# Autodesk Inventor assembly: V2 - Full Assembly
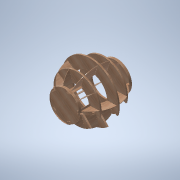
[picture p0: Inventor's stored thumbnail of the model, 180x180]
Saved by Autodesk Inventor 2021 (Build 250183000, 183)
## iProperties
Created: 2020-07-30
Part Number: V2 - Full Assembly
Document SubType Name: Assembly
Designer: Dan Wikman
Author: Dan Wikman
## Documents named in this file (17)
- C:\Users\danny\OneDrive\University Life\2020, Semester 1\METR4900 Honours Thesis\PROTOTYPE V2\V2 - Full Assembly.iam
- C:\Users\danny\OneDrive\University Life\2020, Semester 1\METR4900 Honours Thesis\PROTOTYPE V2\Base - V2.ipt
- C:\Users\danny\OneDrive\University Life\2020, Semester 1\METR4900 Honours Thesis\PROTOTYPE V2\Vertical Support Assembly.iam
- C:\Users\danny\OneDrive\University Life\2020, Semester 1\METR4900 Honours Thesis\PROTOTYPE V2\Support A1 - V2.ipt
- C:\Users\danny\OneDrive\University Life\2020, Semester 1\METR4900 Honours Thesis\PROTOTYPE V2\Level 1 Support Ends.ipt
- C:\Users\danny\OneDrive\University Life\2020, Semester 1\METR4900 Honours Thesis\PROTOTYPE V2\Level 1 Support Mid.ipt
- C:\Users\danny\OneDrive\University Life\2020, Semester 1\METR4900 Honours Thesis\PROTOTYPE V2\Level 1 Ring Assembly.iam
- C:\Users\danny\OneDrive\University Life\2020, Semester 1\METR4900 Honours Thesis\PROTOTYPE V2\Level 3 Assembly.iam
- C:\Users\danny\OneDrive\University Life\2020, Semester 1\METR4900 Honours Thesis\PROTOTYPE V2\Level 2 Ring Assembly.iam
- C:\Users\danny\OneDrive\University Life\2020, Semester 1\METR4900 Honours Thesis\PROTOTYPE V2\Roof - V2.ipt
- C:\Users\danny\OneDrive\University Life\2020, Semester 1\METR4900 Honours Thesis\PROTOTYPE V2\Level 2 Edge Banding.ipt
- C:\Users\danny\OneDrive\University Life\2020, Semester 1\METR4900 Honours Thesis\PROTOTYPE V2\Level 1 Edge Banding.ipt
- C:\Users\danny\OneDrive\University Life\2020, Semester 1\METR4900 Honours Thesis\PROTOTYPE V2\Roof Banding.ipt
- C:\Users\danny\OneDrive\University Life\2020, Semester 1\METR4900 Honours Thesis\PROTOTYPE V2\Floor Banding.ipt
- C:\Users\danny\OneDrive\University Life\2020, Semester 1\METR4900 Honours Thesis\PROTOTYPE V2\Wedge Assembly.iam
- C:\Users\danny\OneDrive\University Life\2020, Semester 1\METR4900 Honours Thesis\PROTOTYPE V2\Feet - V2.ipt
- C:\Users\danny\OneDrive\University Life\2020, Semester 1\METR4900 Honours Thesis\PROTOTYPE V2\Level 3 Edge Banding.ipt
## Components (47 placed, 16 different names)
1. Base - V2:1 — Mate:3, Mate:7, Mate:8, Mate:9, Mate:17, Mate:18, Mate:20, Mate:21, Mate:22, Mate:25, Mate:55, Mate:56, Mate:57, Mate:58, Mate:60
2. Level 1 Support Ends:1 — Mate:16, Mate:17, Mate:18
3. Level 1 Support Ends:2 — Mate:19, Mate:20, Mate:21
4. Level 1 Ring Assembly:1 [sub-assembly] — Mate:31, Mate:32, Mate:33, Mate:47, Mate:48
5. Level 2 Ring Assembly:1 [sub-assembly] — Mate:38, Mate:43, Mate:44, Mate:45, Mate:46, Flush:1
6. Level 3 Assembly:2 [sub-assembly] — Mate:34, Mate:63, Mate:64, Mate:65, Mate:66
7. Roof - V2:1 — Mate:40, Mate:41, Mate:42, Mate:53
8. Level 2 Edge Banding:1 — Mate:45, Mate:46, Flush:1
9. Level 1 Edge Banding:1 — Mate:47, Mate:48, Mate:49
10. Roof Banding:1 — Mate:53, Flush:2
11. Floor Banding:1 — Mate:57, Flush:3
12. Level 3 Edge Banding:1 — Mate:65, Mate:66, Mate:67
13. Vertical Support Assembly:1 [sub-assembly] — Mate:3, Mate:32, Mate:34, Mate:38, Mate:41, Mate:42, Mate:43, Mate:44, Mate:55, Mate:56, Mate:63, Mate:64
14. Vertical Support Assembly:2 [sub-assembly]
15. Vertical Support Assembly:3 [sub-assembly] — Mate:16, Mate:33, Mate:49, Flush:2, Flush:3, Mate:59, Flush:4, Mate:61, Mate:62
16. Vertical Support Assembly:4 [sub-assembly] — Mate:19, Mate:31
17. Vertical Support Assembly:5 [sub-assembly] — Mate:23, Mate:24, Mate:26, Mate:27, Mate:40, Mate:67
18. Support A1 - V2:1 — Mate:7, Mate:9
19. Support A1 - V2:2 — Mate:8
20. Support A1 - V2:3
21. Support A1 - V2:4
22. Level 1 Support Mid:1 — Mate:22, Mate:23, Mate:24
23. Level 1 Support Mid:2 — Mate:25, Mate:26, Mate:27
24. Level 1 Support Mid:3
25. Level 1 Support Mid:4
26. Level 1 Support Mid:5
27. Level 1 Support Mid:6
28. Wedge Assembly:1 [sub-assembly] — Mate:58, Mate:59, Flush:4
29. Wedge Assembly:2 [sub-assembly]
30. Wedge Assembly:3 [sub-assembly]
31. Wedge Assembly:4 [sub-assembly]
32. Wedge Assembly:5 [sub-assembly]
33. Feet - V2:1 — Mate:60, Mate:61, Mate:62
34. Feet - V2:2
35. Feet - V2:3
36. Feet - V2:4
37. Feet - V2:5
38. Feet - V2:6
39. Feet - V2:7
40. Feet - V2:8
41. Feet - V2:9
42. Feet - V2:10
43. Feet - V2:11
44. Feet - V2:12
45. Feet - V2:13
46. Feet - V2:14
47. Feet - V2:15
## Component patterns: (5 elements, first: Vertical Support Assembly:1), (4 elements, first: Support A1 - V2:1), (3 elements, first: Level 1 Support Mid:1 + Level 1 Support Mid:2), (5 elements, first: Wedge Assembly:1), (5 elements), (3 elements, first: Feet - V2:1), Component Pattern 5:2 (3 elements), Component Pattern 5:3 (3 elements), Component Pattern 5:4 (3 elements), Component Pattern 5:5 (3 elements)
## Relationships (49: Mate 45, Flush 4)
- Mate:3 (0.25 mm): Base - V2:1 ↔ Vertical Support Assembly:1
- Mate:7 (0.25 mm): Base - V2:1 ↔ Support A1 - V2:1
- Mate:8: Base - V2:1 ↔ Support A1 - V2:2
- Mate:9 (1.75 mm): Base - V2:1 ↔ Support A1 - V2:1
- Mate:16: Level 1 Support Ends:1 ↔ Vertical Support Assembly:3
- Mate:17: Base - V2:1 ↔ Level 1 Support Ends:1
- Mate:18 (0.25 mm): Base - V2:1 ↔ Level 1 Support Ends:1
- Mate:19: Level 1 Support Ends:2 ↔ Vertical Support Assembly:4
- Mate:20: Base - V2:1 ↔ Level 1 Support Ends:2
- Mate:21 (0.25 mm): Base - V2:1 ↔ Level 1 Support Ends:2
- Mate:22: Base - V2:1 ↔ Level 1 Support Mid:1
- Mate:23: Vertical Support Assembly:5 ↔ Level 1 Support Mid:1
- Mate:24 (0.25 mm): Vertical Support Assembly:5 ↔ Level 1 Support Mid:1
- Mate:25: Base - V2:1 ↔ Level 1 Support Mid:2
- Mate:26 (0.25 mm): Vertical Support Assembly:5 ↔ Level 1 Support Mid:2
- Mate:27: Vertical Support Assembly:5 ↔ Level 1 Support Mid:2
- Mate:31: Level 1 Ring Assembly:1 ↔ Vertical Support Assembly:4
- Mate:32 (0.25 mm): Level 1 Ring Assembly:1 ↔ Vertical Support Assembly:1
- Mate:33 (0.25 mm): Level 1 Ring Assembly:1 ↔ Vertical Support Assembly:3
- Mate:34: Level 3 Assembly:2 ↔ Vertical Support Assembly:1
- Mate:38: Level 2 Ring Assembly:1 ↔ Vertical Support Assembly:1
- Mate:40: Roof - V2:1 ↔ Vertical Support Assembly:5
- Mate:41 (0.25 mm): Roof - V2:1 ↔ Vertical Support Assembly:1
- Mate:42 (1.75 mm): Roof - V2:1 ↔ Vertical Support Assembly:1
- Mate:43 (1.75 mm): Level 2 Ring Assembly:1 ↔ Vertical Support Assembly:1
- Mate:44 (0.25 mm): Level 2 Ring Assembly:1 ↔ Vertical Support Assembly:1
- Mate:45: Level 2 Ring Assembly:1 ↔ Level 2 Edge Banding:1
- Mate:46: Level 2 Ring Assembly:1 ↔ Level 2 Edge Banding:1
- Flush:1: Level 2 Ring Assembly:1 ↔ Level 2 Edge Banding:1
- Mate:47: Level 1 Ring Assembly:1 ↔ Level 1 Edge Banding:1
- Mate:48: Level 1 Ring Assembly:1 ↔ Level 1 Edge Banding:1
- Mate:49: Level 1 Edge Banding:1 ↔ Vertical Support Assembly:3
- Mate:53: Roof - V2:1 ↔ Roof Banding:1
- Flush:2: Roof Banding:1 ↔ Vertical Support Assembly:3
- Mate:55: Base - V2:1 ↔ Vertical Support Assembly:1
- Mate:56 (1.75 mm): Base - V2:1 ↔ Vertical Support Assembly:1
- Mate:57: Base - V2:1 ↔ Floor Banding:1
- Flush:3: Floor Banding:1 ↔ Vertical Support Assembly:3
- Mate:58: Base - V2:1 ↔ Wedge Assembly:1
- Mate:59 (0.25 mm): Vertical Support Assembly:3 ↔ Wedge Assembly:1
- Flush:4 (-24.355 mm): Vertical Support Assembly:3 ↔ Wedge Assembly:1
- Mate:60: Base - V2:1 ↔ Feet - V2:1
- Mate:61 (2.5 mm): Vertical Support Assembly:3 ↔ Feet - V2:1
- Mate:62 (0.25 mm): Vertical Support Assembly:3 ↔ Feet - V2:1
- Mate:63 (1.75 mm): Level 3 Assembly:2 ↔ Vertical Support Assembly:1
- Mate:64 (0.25 mm): Level 3 Assembly:2 ↔ Vertical Support Assembly:1
- Mate:65: Level 3 Assembly:2 ↔ Level 3 Edge Banding:1
- Mate:66: Level 3 Assembly:2 ↔ Level 3 Edge Banding:1
- Mate:67: Level 3 Edge Banding:1 ↔ Vertical Support Assembly:5
